# Autodesk Inventor assembly: Shooter Assembly
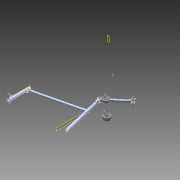
[picture p0: Inventor's stored thumbnail of the model, 180x180]
Saved by Autodesk Inventor 2014 (Build 180170000, 170)
## iProperties
Created: 2014-01-05
Part Number: Shooter Assembly
Document SubType Name: Assembly
Designer: Andrew Toennies
Mass: 930.3 g
Surface Area: 4612.02 cm^2
Volume: 294.178 cm^3
Density: 3.16237 g/cm^3
Author: Andrew Toennies
## Documents named in this file (19)
- C:\Users\Andrew Toennies\Documents\GitHub\2014buildCAD\Shooter\Shooter Assembly.iam
- C:\Users\Andrew Toennies\Documents\GitHub\2014buildCAD\Shooter\Vex Pro 1x1 rectangular tubing 12 in length.ipt
- C:\Users\Andrew Toennies\Documents\GitHub\2014buildCAD\Shooter\Vex Pro End Bearing Mount.ipt
- C:\Users\Andrew Toennies\Documents\GitHub\2014buildCAD\Shooter\Vex Pro 1x1 rectangular tubing 27 in length.ipt
- C:\Users\Andrew Toennies\Documents\GitHub\2014buildCAD\Shooter\Vex Pro 1x1 rectangular tubing 24 in length.ipt
- C:\Users\Andrew Toennies\Documents\GitHub\2014buildCAD\Shooter\Vex Pro T gusset.ipt
- C:\Users\Andrew Toennies\Documents\GitHub\2014buildCAD\Shooter\Vex Pro Corner Gusset.ipt
- C:\Users\Andrew Toennies\Documents\GitHub\2014buildCAD\Shooter\Vex Pro 1x1 rectangular tubing 13 in length.ipt
- C:\Users\Andrew Toennies\Documents\GitHub\2014buildCAD\Shooter\Vex Pro Side Bearing Gusset.ipt
- C:\Users\Andrew Toennies\Documents\GitHub\2014buildCAD\Shooter\Bearing ID 0.500 Hex OD 1.125.ipt
- C:\Users\Andrew Toennies\Documents\GitHub\2014buildCAD\Shooter\Axle 0.500 Hex 5 in length.ipt
- C:\Users\Andrew Toennies\Documents\GitHub\2014buildCAD\Shooter\Spacer.ipt
- C:\Users\Andrew Toennies\Documents\GitHub\2014buildCAD\Shooter\Bearing ID 0.375 OD 1.125.ipt
- C:\Users\Andrew Toennies\Documents\GitHub\2014buildCAD\Shooter\Axle 0.375 3 in length.ipt
- C:\Users\Andrew Toennies\Documents\GitHub\2014buildCAD\Shooter\Vex Pro 18 tooth timing belt pulley.ipt
- C:\Users\Andrew Toennies\Documents\GitHub\2014buildCAD\Shooter\Vex Pro 30 tooth 9mm timing belt pulley.ipt
- C:\Users\Andrew Toennies\Documents\GitHub\2014buildCAD\Shooter\Vex Pro Traction Wheel 4 in dia 1.5 in wide.iam
- C:\Users\Andrew Toennies\Documents\GitHub\2014buildCAD\Shooter\Vex Pro Traction Wheel 4 in dia 1 in wide.iam
- C:\Users\Andrew Toennies\Documents\GitHub\2014buildCAD\Shooter\Vex Pro VersaHub 0.500 Hex.ipt
## Components (32 placed, 18 different names)
1. Vex Pro 1x1 rectangular tubing 12 in length:1 — Flush:1, Insert:9, Insert:10, Insert:11, Insert:12, Insert:17, Insert:18, Insert:19, Insert:20, Flush:4
2. Vex Pro 1x1 rectangular tubing 27 in length:1 — Flush:1, Insert:5, Insert:6, Insert:7, Insert:8, Flush:2, Mate:2, Mate:5
3. Vex Pro 1x1 rectangular tubing 24 in length:1 — Flush:2, Mate:2, Flush:3, Mate:6, Insert:27, Insert:28, Insert:31, Insert:32, Flush:9
4. Vex Pro T gusset:1 — Insert:5, Insert:6, Mate:6
5. Vex Pro T gusset:2 — Insert:7, Insert:8
6. Vex Pro Corner Gusset:1 — Insert:9, Insert:10, Flush:6
7. Vex Pro Corner Gusset:2 — Insert:11, Insert:12
8. Vex Pro End Bearing Mount:3 — Insert:29, Insert:30, Insert:35
9. Vex Pro End Bearing Mount:4 — Mate:4, Insert:33, Insert:34, Insert:36
10. Vex Pro 1x1 rectangular tubing 13 in length:1 — Mate:4, Flush:3, Insert:21, Insert:22, Insert:23, Insert:24, Flush:8
11. Vex Pro End Bearing Mount:5 — Insert:21, Insert:22, Insert:25
12. Vex Pro End Bearing Mount:6 — Insert:23, Insert:24, Insert:26
13. Vex Pro Side Bearing Gusset:1 — Insert:17, Insert:18, Insert:37
14. Vex Pro Side Bearing Gusset:2 — Insert:19, Insert:20, Mate:5, Insert:38
15. Bearing ID 0.500 Hex OD 1.125:1 — Insert:26, Flush:7, Mate:7, Mate:8
16. Bearing ID 0.500 Hex OD 1.125:2 — Insert:25, Flush:7, Mate:10, Mate:16
17. Axle 0.500 Hex 5 in length:1 — Mate:7, Mate:8, Flush:8, Flush:10, Flush:11, Mate:14, Mate:15
18. Spacer:1 — Insert:31, Insert:32, Insert:33, Insert:34
19. Spacer:2 — Insert:27, Insert:28, Insert:29, Insert:30
20. Bearing ID 0.375 OD 1.125:1 — Insert:35, Mate:9
21. Bearing ID 0.375 OD 1.125:2 — Insert:36
22. Axle 0.375 3 in length:1 — Mate:9, Flush:9, Mate:13
23. Vex Pro 18 tooth timing belt pulley:1
24. Vex Pro 30 tooth 9mm timing belt pulley:1 — Mate:14, Mate:15, Mate:16
25. Bearing ID 0.375 OD 1.125:3 — Insert:37
26. Bearing ID 0.375 OD 1.125:4 — Insert:38
27. Vex Pro Traction Wheel 4 in dia 1.5 in wide:1 [sub-assembly]
28. Vex Pro Traction Wheel 4 in dia 1 in wide:1 [sub-assembly]
29. Vex Pro VersaHub 0.500 Hex:1
30. Vex Pro VersaHub 0.500 Hex:2
31. Vex Pro VersaHub 0.500 Hex:3
32. Vex Pro VersaHub 0.500 Hex:4
## Relationships (55: Insert 30, Mate 14, Flush 11)
- Flush:1: Vex Pro 1x1 rectangular tubing 12 in length:1 ↔ Vex Pro 1x1 rectangular tubing 27 in length:1
- Insert:5: Vex Pro 1x1 rectangular tubing 27 in length:1 ↔ Vex Pro T gusset:1
- Insert:6: Vex Pro 1x1 rectangular tubing 27 in length:1 ↔ Vex Pro T gusset:1
- Insert:7: Vex Pro 1x1 rectangular tubing 27 in length:1 ↔ Vex Pro T gusset:2
- Insert:8: Vex Pro 1x1 rectangular tubing 27 in length:1 ↔ Vex Pro T gusset:2
- Flush:2: Vex Pro 1x1 rectangular tubing 27 in length:1 ↔ Vex Pro 1x1 rectangular tubing 24 in length:1
- Mate:2: Vex Pro 1x1 rectangular tubing 27 in length:1 ↔ Vex Pro 1x1 rectangular tubing 24 in length:1
- Insert:9: Vex Pro 1x1 rectangular tubing 12 in length:1 ↔ Vex Pro Corner Gusset:1
- Insert:10: Vex Pro 1x1 rectangular tubing 12 in length:1 ↔ Vex Pro Corner Gusset:1
- Insert:11: Vex Pro 1x1 rectangular tubing 12 in length:1 ↔ Vex Pro Corner Gusset:2
- Insert:12: Vex Pro 1x1 rectangular tubing 12 in length:1 ↔ Vex Pro Corner Gusset:2
- Mate:4: Vex Pro End Bearing Mount:4 ↔ Vex Pro 1x1 rectangular tubing 13 in length:1
- Flush:3: Vex Pro 1x1 rectangular tubing 24 in length:1 ↔ Vex Pro 1x1 rectangular tubing 13 in length:1
- Insert:17: Vex Pro 1x1 rectangular tubing 12 in length:1 ↔ Vex Pro Side Bearing Gusset:1
- Insert:18: Vex Pro 1x1 rectangular tubing 12 in length:1 ↔ Vex Pro Side Bearing Gusset:1
- Insert:19: Vex Pro 1x1 rectangular tubing 12 in length:1 ↔ Vex Pro Side Bearing Gusset:2
- Insert:20: Vex Pro 1x1 rectangular tubing 12 in length:1 ↔ Vex Pro Side Bearing Gusset:2
- Mate:5: Vex Pro 1x1 rectangular tubing 27 in length:1 ↔ Vex Pro Side Bearing Gusset:2
- Flush:4: Vex Pro 1x1 rectangular tubing 12 in length:1
- Mate:6: Vex Pro 1x1 rectangular tubing 24 in length:1 ↔ Vex Pro T gusset:1
- Flush:5 (-711.2 mm)
- Flush:6 (-1422.4 mm): Vex Pro Corner Gusset:1
- Insert:21: Vex Pro 1x1 rectangular tubing 13 in length:1 ↔ Vex Pro End Bearing Mount:5
- Insert:22: Vex Pro 1x1 rectangular tubing 13 in length:1 ↔ Vex Pro End Bearing Mount:5
- Insert:23: Vex Pro 1x1 rectangular tubing 13 in length:1 ↔ Vex Pro End Bearing Mount:6
- Insert:24: Vex Pro 1x1 rectangular tubing 13 in length:1 ↔ Vex Pro End Bearing Mount:6
- Insert:25: Vex Pro End Bearing Mount:5 ↔ Bearing ID 0.500 Hex OD 1.125:2
- Insert:26: Vex Pro End Bearing Mount:6 ↔ Bearing ID 0.500 Hex OD 1.125:1
- Flush:7: Bearing ID 0.500 Hex OD 1.125:1 ↔ Bearing ID 0.500 Hex OD 1.125:2
- Mate:7: Bearing ID 0.500 Hex OD 1.125:1 ↔ Axle 0.500 Hex 5 in length:1
- Mate:8: Bearing ID 0.500 Hex OD 1.125:1 ↔ Axle 0.500 Hex 5 in length:1
- Flush:8 (-50.8 mm): Vex Pro 1x1 rectangular tubing 13 in length:1 ↔ Axle 0.500 Hex 5 in length:1
- Insert:27: Vex Pro 1x1 rectangular tubing 24 in length:1 ↔ Spacer:2
- Insert:28: Vex Pro 1x1 rectangular tubing 24 in length:1 ↔ Spacer:2
- Insert:29: Vex Pro End Bearing Mount:3 ↔ Spacer:2
- Insert:30: Vex Pro End Bearing Mount:3 ↔ Spacer:2
- Insert:31: Vex Pro 1x1 rectangular tubing 24 in length:1 ↔ Spacer:1
- Insert:32: Vex Pro 1x1 rectangular tubing 24 in length:1 ↔ Spacer:1
- Insert:33: Vex Pro End Bearing Mount:4 ↔ Spacer:1
- Insert:34: Vex Pro End Bearing Mount:4 ↔ Spacer:1
- Insert:35: Vex Pro End Bearing Mount:3 ↔ Bearing ID 0.375 OD 1.125:1
- Insert:36: Vex Pro End Bearing Mount:4 ↔ Bearing ID 0.375 OD 1.125:2
- Mate:9: Bearing ID 0.375 OD 1.125:1 ↔ Axle 0.375 3 in length:1
- Flush:9 (-25.4 mm): Vex Pro 1x1 rectangular tubing 24 in length:1 ↔ Axle 0.375 3 in length:1
- Mate:10: Bearing ID 0.500 Hex OD 1.125:2
- Flush:10 (-4.7625 mm): Axle 0.500 Hex 5 in length:1
- Flush:11 (-4.7625 mm): Axle 0.500 Hex 5 in length:1
- Mate:11
- Mate:12
- Mate:13: Axle 0.375 3 in length:1
- Mate:14: Axle 0.500 Hex 5 in length:1 ↔ Vex Pro 30 tooth 9mm timing belt pulley:1
- Mate:15: Axle 0.500 Hex 5 in length:1 ↔ Vex Pro 30 tooth 9mm timing belt pulley:1
- Insert:37: Vex Pro Side Bearing Gusset:1 ↔ Bearing ID 0.375 OD 1.125:3
- Insert:38: Vex Pro Side Bearing Gusset:2 ↔ Bearing ID 0.375 OD 1.125:4
- Mate:16: Bearing ID 0.500 Hex OD 1.125:2 ↔ Vex Pro 30 tooth 9mm timing belt pulley:1
